# Autodesk Inventor assembly: 2018RobotRhinoTrackWithRevLift
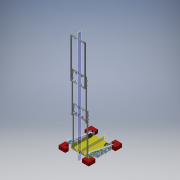
[picture p0: Inventor's stored thumbnail of the model, 180x180]
Saved by Autodesk Inventor 2019 (Build 230136000, 136)
## iProperties
Created: 2017-01-12
Part Number: 2018RobotRhinoTrackWithRevLift
Document SubType Name: Assembly
Designer: steele
Mass: 784427 g
Surface Area: 99187.8 cm^2
Volume: 668402 cm^3
Density: 1.17359 g/cm^3
Author: steele
## Documents named in this file (8)
- D:\snobotics\CAD-Development\robSteele\2018PostSeasonLift\2018RobotRhinoTrackWithRevLift.iam
- D:\snobotics\CAD-Development\robSteele\SnoBotics2017\LeftRhinoTrackAM-3322\am-3322_Rhino_Track_Drive_Module_Left.iam
- D:\snobotics\CAD-Development\robSteele\SnoBotics2017\robotVolume.ipt
- D:\snobotics\CAD-Development\robSteele\SnoBotics2017\RedBumper.ipt
- D:\snobotics\CAD-Development\robSteele\2017CompetitionRobot\Design Accelerator\Bolted Connection1.iam
- D:\snobotics\CAD-Development\robSteele\2018PostSeasonLift\SheetBottomFloor.ipt
- D:\snobotics\CAD-Development\robSteele\2018PostSeasonLift\am-3322_Rhino_Track_Drive_Module_Right.iam
- D:\snobotics\CAD-Development\robSteele\2018PostSeasonLift\TwoStageRev-25-1238-1239.iam
## Components (10 placed, 7 different names)
1. am-3322_Rhino_Track_Drive_Module_Left:1 [sub-assembly] — Flush:3, Flush:4, Flush:5, Mate:3, Flush:20, Flush:21, Mate:5, Flush:22, Flush:23
2. robotVolume:1 — Flush:3, Flush:4, Flush:5, Flush:14, Flush:15, Flush:18, Flush:19
3. RedBumper:1 — Mate:3
4. RedBumper:2
5. RedBumper:3 — Flush:14, Flush:15
6. RedBumper:4 — Flush:18, Flush:19
7. SheetBottomFloor:1 — Flush:20, Flush:21, Mate:5, Mate:6, Mate:7, Flush:24, Flush:25
8. Bolted Connection:1 [sub-assembly]
9. am-3322_Rhino_Track_Drive_Module_Right:1 [sub-assembly] — Mate:6, Flush:22, Flush:23
10. TwoStageRev-25-1238-1239:1 [sub-assembly] — Mate:7, Flush:24, Flush:25
## Relationships (17: Flush 13, Mate 4)
- Flush:3: am-3322_Rhino_Track_Drive_Module_Left:1 ↔ robotVolume:1
- Flush:4 (106.3752 mm): am-3322_Rhino_Track_Drive_Module_Left:1 ↔ robotVolume:1
- Flush:5 (101.6 mm): am-3322_Rhino_Track_Drive_Module_Left:1 ↔ robotVolume:1
- Mate:3: am-3322_Rhino_Track_Drive_Module_Left:1 ↔ RedBumper:1
- Flush:14: robotVolume:1 ↔ RedBumper:3
- Flush:15: robotVolume:1 ↔ RedBumper:3
- Flush:18: robotVolume:1 ↔ RedBumper:4
- Flush:19: robotVolume:1 ↔ RedBumper:4
- Flush:20: am-3322_Rhino_Track_Drive_Module_Left:1 ↔ SheetBottomFloor:1
- Flush:21: am-3322_Rhino_Track_Drive_Module_Left:1 ↔ SheetBottomFloor:1
- Mate:5: am-3322_Rhino_Track_Drive_Module_Left:1 ↔ SheetBottomFloor:1
- Mate:6: SheetBottomFloor:1 ↔ am-3322_Rhino_Track_Drive_Module_Right:1
- Flush:22: am-3322_Rhino_Track_Drive_Module_Left:1 ↔ am-3322_Rhino_Track_Drive_Module_Right:1
- Flush:23: am-3322_Rhino_Track_Drive_Module_Left:1 ↔ am-3322_Rhino_Track_Drive_Module_Right:1
- Mate:7: SheetBottomFloor:1 ↔ TwoStageRev-25-1238-1239:1
- Flush:24: SheetBottomFloor:1 ↔ TwoStageRev-25-1238-1239:1
- Flush:25: SheetBottomFloor:1 ↔ TwoStageRev-25-1238-1239:1
